# Autodesk Inventor assembly: CrossRollerBearingUnit
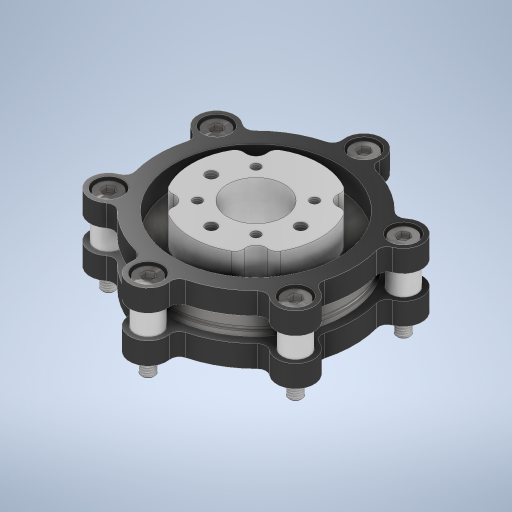
[picture p0: Inventor's stored thumbnail of the model, 512x512]
Saved by Autodesk Inventor 2024.2 (Build 282272000, 272)
## iProperties
Created: 2024-01-04
Part Number: CrossRollerBearingUnit
Document SubType Name: Assembly
Designer: Masato Kubotera
Mass: 106.357 g
Surface Area: 198.931 cm^2
Volume: 22.6759 cm^3
Density: 4.69031 g/cm^3
Author: Masato Kubotera
## Documents named in this file (11)
- C:\Users\masato\OneDrive - Chiba Institute of Technology\CIT Brains\RoboCup2024\Mechanic\SUSTAINA-OP2-DEV\NativeFiles\Boby\CommonDesignedComponents\CrossRollerBearingUnit\CrossRollerBearingUnit.iam
- C:\Users\masato\OneDrive - Chiba Institute of Technology\CIT Brains\RoboCup2024\Mechanic\SUSTAINA-OP2-DEV\NativeFiles\Boby\CommonDesignedComponents\CrossRollerBearingUnit\CrossRollerBearingOuterFlange.ipt
- C:\Users\masato\OneDrive - Chiba Institute of Technology\CIT Brains\RoboCup2024\Mechanic\SUSTAINA-OP2-DEV\NativeFiles\Boby\CommonDesignedComponents\CrossRollerBearingUnit\CrossRollerBearingOuterSupportStand.ipt
- C:\Users\masato\OneDrive - Chiba Institute of Technology\CIT Brains\RoboCup2024\Mechanic\SUSTAINA-OP2-DEV\NativeFiles\Boby\COTS\Screws\CapScrew\UC-0306.ipt
- C:\Users\masato\OneDrive - Chiba Institute of Technology\CIT Brains\RoboCup2024\Mechanic\SUSTAINA-OP2-DEV\NativeFiles\Boby\COTS\Bearings\RB2508UUC0.ipt
- C:\Users\masato\OneDrive - Chiba Institute of Technology\CIT Brains\RoboCup2024\Mechanic\SUSTAINA-OP2-DEV\NativeFiles\Boby\CommonDesignedComponents\CrossRollerBearingUnit\CrossRollerBearingInnerFlange.ipt
- C:\Users\masato\OneDrive - Chiba Institute of Technology\CIT Brains\RoboCup2024\Mechanic\SUSTAINA-OP2-DEV\NativeFiles\Boby\COTS\Screws\CapScrew\UC-0310.ipt
- C:\Users\masato\OneDrive - Chiba Institute of Technology\CIT Brains\RoboCup2024\Mechanic\SUSTAINA-OP2-DEV\NativeFiles\Boby\CommonDesignedComponents\CrossRollerBearingUnit\CrossRollerBearingInnerSupportStand.ipt
- C:\Users\masato\OneDrive - Chiba Institute of Technology\CIT Brains\RoboCup2024\Mechanic\SUSTAINA-OP2-DEV\NativeFiles\Boby\COTS\Spacers\BRU-309S.ipt
- C:\Users\masato\OneDrive - Chiba Institute of Technology\CIT Brains\RoboCup2024\Mechanic\SUSTAINA-OP2-DEV\NativeFiles\Boby\COTS\Spacers\BRU-307S.ipt
- C:\Users\masato\OneDrive - Chiba Institute of Technology\CIT Brains\RoboCup2024\Mechanic\SUSTAINA-OP2-DEV\NativeFiles\Boby\COTS\Screws\ScrewsWithShoulder\LMSBP4-10.ipt
## Components (23 placed, 10 different names)
1. CrossRollerBearingOuterSupportStand:1 — Flush:1, Flush:2, Flush:3, Insert:1, Insert:2, Insert:6
2. CrossRollerBearingOuterFlange:1 — Insert:3, Insert:4, Insert:5
3. CrossRollerBearingInnerFlange:1 — Insert:7, Angle:4, Insert:12
4. CrossRollerBearingInnerSupportStand:1 — Insert:11, Angle:8
5. UC-0310:1 — Angle:5
6. UC-0310:2 — Angle:6
7. BRU-307S:1 — Insert:1, Angle:1, Insert:4
8. RB2508UUC0:1 — Insert:6, Flush:4, Flush:5, Insert:7, Insert:11
9. BRU-309S:1 — Insert:2, Angle:2, Insert:3
10. BRU-309S:2
11. BRU-309S:3
12. BRU-309S:4
13. BRU-309S:5
14. UC-0306:1 — Insert:5, Angle:3
15. UC-0306:2
16. UC-0306:3
17. UC-0306:4
18. UC-0306:5
19. UC-0306:6
20. LMSBP4-10:1 — Insert:12
21. LMSBP4-10:2
22. LMSBP4-10:3
23. LMSBP4-10:4
## Component patterns: (5 elements, first: BRU-309S:1), (6 elements, first: UC-0306:1), (4 elements, first: LMSBP4-10:1)
## Relationships (21: Insert 9, Angle 7, Flush 5)
- Flush:1: CrossRollerBearingOuterSupportStand:1
- Flush:2: CrossRollerBearingOuterSupportStand:1
- Flush:3: CrossRollerBearingOuterSupportStand:1
- Insert:1: CrossRollerBearingOuterSupportStand:1 ↔ BRU-307S:1
- Insert:2: CrossRollerBearingOuterSupportStand:1 ↔ BRU-309S:1
- Angle:1 (0 deg): BRU-307S:1
- Angle:2 (0 deg): BRU-309S:1
- Insert:3: CrossRollerBearingOuterFlange:1 ↔ BRU-309S:1
- Insert:4: CrossRollerBearingOuterFlange:1 ↔ BRU-307S:1
- Insert:5: CrossRollerBearingOuterFlange:1 ↔ UC-0306:1
- Angle:3 (0 deg): UC-0306:1
- Insert:6: CrossRollerBearingOuterSupportStand:1 ↔ RB2508UUC0:1
- Flush:4: RB2508UUC0:1
- Flush:5: RB2508UUC0:1
- Insert:7: CrossRollerBearingInnerFlange:1 ↔ RB2508UUC0:1
- Angle:4 (0 deg): CrossRollerBearingInnerFlange:1
- Angle:5 (0 deg): UC-0310:1
- Angle:6 (0 deg): UC-0310:2
- Insert:11: CrossRollerBearingInnerSupportStand:1 ↔ RB2508UUC0:1
- Angle:8 (0 deg): CrossRollerBearingInnerSupportStand:1
- Insert:12: CrossRollerBearingInnerFlange:1 ↔ LMSBP4-10:1
